# Autodesk Inventor assembly: ThinkBoard
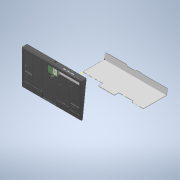
[picture p0: Inventor's stored thumbnail of the model, 180x180]
Saved by Autodesk Inventor 2022 (Build 260153000, 153)
## iProperties
Created: 2021-08-10
Part Number: ThinkBoard
Document SubType Name: Assembly
Designer: Administrator
Title: ThinkBoard v2
Author: Administrator
## Documents named in this file (6)
- C:\Users\benka\Downloads\ThinkBoard v1\ThinkBoard.iam
- C:\Users\benka\Downloads\ThinkBoard v1\USB Hub.ipt
- C:\Users\benka\Downloads\ThinkBoard v1\Case.ipt
- C:\Users\benka\Downloads\ThinkBoard v1\Teensy_3-2 v1.ipt
- C:\Users\benka\Downloads\T420 Backplate Ben.ipt
- C:\Users\benka\Downloads\ThinkBoard v1\Lenovo_Scanner t32.iam
## Components (5 placed, 5 different names)
1. USB Hub:1
2. Case:1 — Mate:1
3. Teensy_3-2 v1:1 — Insert:1
4. T420 Backplate Ben:1
5. Lenovo_Scanner t32:1 [sub-assembly] — Insert:1, Mate:1
## Relationships (2: Insert 1, Mate 1)
- Insert:1 (3 mm): Teensy_3-2 v1:1 ↔ Lenovo_Scanner t32:1
- Mate:1: Case:1 ↔ Lenovo_Scanner t32:1
